# Autodesk Inventor assembly: Assembly1
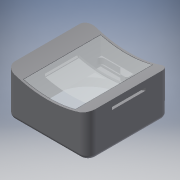
[picture p0: Inventor's stored thumbnail of the model, 180x180]
Saved by Autodesk Inventor 2016 (Build 200138000, 138)
## iProperties
Created: 2016-05-27
Part Number: Assembly1
Document SubType Name: Assembly
Designer: xdlea
Author: xdlea
## Documents named in this file (3)
- D:\Library\Documents\7-Git\SPCN-TrackingBracelet\CAD\Final Revision\Final Track.iam
- D:\Library\Documents\7-Git\SPCN-TrackingBracelet\CAD\Final Revision\Final Track Cover.ipt
- D:\Library\Documents\7-Git\SPCN-TrackingBracelet\CAD\Final Revision\Final Track Body.ipt
## Components (2 placed, 2 different names)
1. Final Track Cover:1 — Mate:1, Mate:2, Mate:3
2. Final Track Body:1 — Mate:1, Mate:2, Mate:3
## Relationships (3: Mate 3)
- Mate:1: Final Track Cover:1 ↔ Final Track Body:1
- Mate:2: Final Track Cover:1 ↔ Final Track Body:1
- Mate:3: Final Track Cover:1 ↔ Final Track Body:1
